# Autodesk Inventor assembly: C-AC0806M
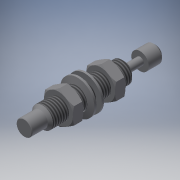
[picture p0: Inventor's stored thumbnail of the model, 180x180]
Saved by Autodesk Inventor 2019 (Build 230136000, 136)
## iProperties
Category: PARTsolutions
Company: MISUMI
Created: 2023-10-14
Part Number: C-AC0806M
Catalog Web Link: www.cadenas.de
Description: C-AC____, C-AC____-N-Economy Shock Absorbers Single-Orifice
Vendor: MISUMI
Document SubType Name: Assembly
Designer: psAdmin
Manufacturer: MISUMI
Mass: 2.63741 g
Surface Area: 26.9097 cm^2
Volume: 2.63741 cm^3
Density: 1 g/cm^3
Title: C-AC0806M
Author: Cadenas PARTsolutions
Comments: Economy Shock Absorbers Single-Orifice
PSOL_IDENT_0: {$CADENAS_DATA/23d-libs/misumi/metric/29_springs/c_ac_____asmtab.prj},191 {VTYP=3D},{STYP=ASSTAB},{N
PSOL_IDENT_1: B=C-AC0806M},{LINA=C-AC0806M},{NN=C-AC____, C-AC____-N},{DATE=28.09.2022 01:02:07},{GEOMDATE=19.05.2
PSOL_IDENT_2: 022 01:59:23},{VERSION=},{LINEID=180},{WBVAR=TS,V},{WBNUMERIC=}  {NB=C-AC0806M},{LINA=C-AC0806M},{KT=
PSOL_IDENT_3: DUMMY},{PN=C-AC0806M},{TYPE=C-AC0806M},{TS=Cap},{TSALG= 'Cap','Cap','No Cap','No Cap' },{NO=0806},{V=
PSOL_IDENT_4: M},{M=M8x1.0},{M3D=8},{PITCH=1.00},{S=6},{L=50.0},{L1=32.0},{L2=6.0},{T=4.0},{TT=6.0},{DD=6.6},{DD1=
PSOL_IDENT_5: 2.9},{B=11.0},{LW=With},{LW1=15.0},{LW2=17.0},{NUT1=7.000},{NUT2=23.000},{C3D=6.000},{L3=20},{PPATH=
PSOL_IDENT_6: c_ac____/c_ac_____asmtpl.prj}
NB: C-AC0806M
NN: C-AC____, C-AC____-N
NT: Economy Shock Absorbers Single-Orifice
NBSYN: $PN.
LINA: C-AC0806M
CATALOG: Misumi
PN: C-AC0806M
TS: Cap
NO: 0806
V: M
M: M8x1.0
S: 6
L: 50
L1: 32
L2: 6
T: 4
TT: 6
DD: 6.6
DD1: 2.9
B: 11
LW: With
SUPPLIER: MISUMI
ARTICLENO: C-AC0806M
BOMINFO: C-AC0806M
CREATOR: CADENAS GmbH
## Documents named in this file (5)
- e:\temp\worker_COMMON_2\temp\tmp_2264_132_1cOQU\format_0\C-AC0806M.iam
- e:\temp\worker_COMMON_2\temp\tmp_2264_132_1cOQU\format_0\C-AC0806M_b.ipt
- e:\temp\worker_COMMON_2\temp\tmp_2264_132_1cOQU\format_0\C-AC0806-nut_n.ipt
- e:\temp\worker_COMMON_2\temp\tmp_2264_132_1cOQU\format_0\C-AC-WASHERS-M8.ipt
- e:\temp\worker_COMMON_2\temp\tmp_2264_132_1cOQU\format_0\C-AC0806_r.ipt
## Components (6 placed, 4 different names)
1. C-AC0806M_b:1 — to_nut1_Z@1 <-> to_body1_Z@2, to_nut1_YZ@1 <-> to_body1_YZ@2, to_nut2_Z@1 <-> to_body2_Z@3, to_nut2_YZ@1 <-> to_body2_YZ@3, to_washers_1_Z@1 <-> to_body1_Z@4, to_washers_1_YZ@1 <-> to_body1_YZ@4, to_washers_2_Z@1 <-> to_bolt2_Z@5, to_washers_2_YZ@1 <-> to_bolt2_YZ@5, to_rod_Z@1 <-> to_body_Z@6, to_rod_YZ@1 <-> to_body_YZ@6
2. C-AC0806-nut_n:1 — to_nut1_Z@1 <-> to_body1_Z@2, to_nut1_YZ@1 <-> to_body1_YZ@2
3. C-AC0806-nut_n:2 — to_nut2_Z@1 <-> to_body2_Z@3, to_nut2_YZ@1 <-> to_body2_YZ@3
4. C-AC-WASHERS-M8:1 — to_washers_1_Z@1 <-> to_body1_Z@4, to_washers_1_YZ@1 <-> to_body1_YZ@4
5. C-AC-WASHERS-M8:2 — to_washers_2_Z@1 <-> to_bolt2_Z@5, to_washers_2_YZ@1 <-> to_bolt2_YZ@5
6. C-AC0806_r:1 — to_rod_Z@1 <-> to_body_Z@6, to_rod_YZ@1 <-> to_body_YZ@6
## Relationships (10: Mate 5, Angle 5)
- to_nut1_Z@1 <-> to_body1_Z@2 [Mate]: C-AC0806M_b:1 ↔ C-AC0806-nut_n:1
- to_nut1_YZ@1 <-> to_body1_YZ@2 [Angle] (0 deg): C-AC0806M_b:1 ↔ C-AC0806-nut_n:1
- to_nut2_Z@1 <-> to_body2_Z@3 [Mate]: C-AC0806M_b:1 ↔ C-AC0806-nut_n:2
- to_nut2_YZ@1 <-> to_body2_YZ@3 [Angle] (0 deg): C-AC0806M_b:1 ↔ C-AC0806-nut_n:2
- to_washers_1_Z@1 <-> to_body1_Z@4 [Mate]: C-AC0806M_b:1 ↔ C-AC-WASHERS-M8:1
- to_washers_1_YZ@1 <-> to_body1_YZ@4 [Angle] (0 deg): C-AC0806M_b:1 ↔ C-AC-WASHERS-M8:1
- to_washers_2_Z@1 <-> to_bolt2_Z@5 [Mate]: C-AC0806M_b:1 ↔ C-AC-WASHERS-M8:2
- to_washers_2_YZ@1 <-> to_bolt2_YZ@5 [Angle] (0 deg): C-AC0806M_b:1 ↔ C-AC-WASHERS-M8:2
- to_rod_Z@1 <-> to_body_Z@6 [Mate]: C-AC0806M_b:1 ↔ C-AC0806_r:1
- to_rod_YZ@1 <-> to_body_YZ@6 [Angle] (0 deg): C-AC0806M_b:1 ↔ C-AC0806_r:1
